# Autodesk Inventor assembly: Assembly1
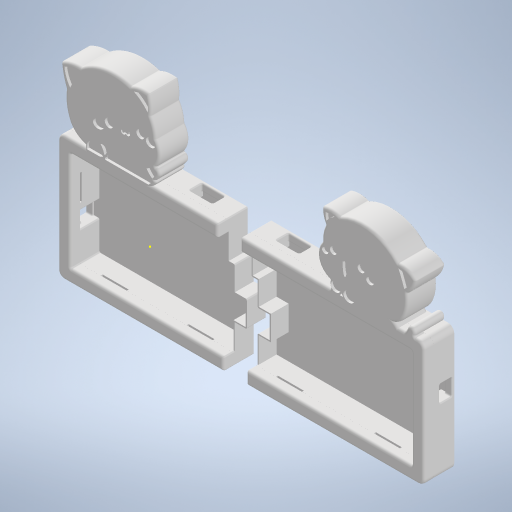
[picture p0: Inventor's stored thumbnail of the model, 512x512]
Saved by Autodesk Inventor 2023 (Build 270158000, 158)
## iProperties
Created: 2022-11-13
Part Number: Assembly1
Document SubType Name: Assembly
Designer: reide
Author: reide
## Documents named in this file (5)
- C:\Users\reide\OneDrive\Documents\Inventor\Fourier Keyboared Case\Top Themes\Peach and Goma\Assembly1.iam
- C:\Users\reide\OneDrive\Documents\Inventor\Fourier Keyboared Case\Mid_Left.ipt
- C:\Users\reide\OneDrive\Documents\Inventor\Fourier Keyboared Case\Mid_Right.ipt
- C:\Users\reide\OneDrive\Documents\Inventor\Fourier Keyboared Case\Top Themes\Peach and Goma\Goma\Goma_Top_Left.ipt
- C:\Users\reide\OneDrive\Documents\Inventor\Fourier Keyboared Case\Top Themes\Peach and Goma\Peach\Peach_Top_Right.ipt
## Components (4 placed, 4 different names)
1. Mid_Left:1 — Flush:1, Flush:2, Flush:3, Flush:4, Mate:1
2. Mid_Right:1 — Flush:1, Flush:2, Flush:5, Flush:6, Mate:2
3. Goma_Top_Left:1 — Flush:3, Flush:4, Mate:1
4. Peach_Top_Right:1 — Flush:5, Flush:6, Mate:2
## Relationships (8: Flush 6, Mate 2)
- Flush:1: Mid_Left:1 ↔ Mid_Right:1
- Flush:2: Mid_Left:1 ↔ Mid_Right:1
- Flush:3: Mid_Left:1 ↔ Goma_Top_Left:1
- Flush:4: Mid_Left:1 ↔ Goma_Top_Left:1
- Mate:1: Mid_Left:1 ↔ Goma_Top_Left:1
- Flush:5: Mid_Right:1 ↔ Peach_Top_Right:1
- Flush:6: Mid_Right:1 ↔ Peach_Top_Right:1
- Mate:2: Mid_Right:1 ↔ Peach_Top_Right:1
